# Autodesk Inventor assembly: Jar Jar
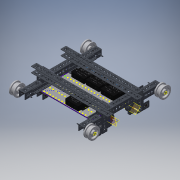
[picture p0: Inventor's stored thumbnail of the model, 180x180]
Saved by Autodesk Inventor 2016 (Build 200138000, 138)
## iProperties
Created: 2015-12-13
Part Number: Jar Jar
Document SubType Name: Assembly
Designer: tbloo
Author: tbloo
## Documents named in this file (17)
- C:\Users\TimB\Documents\GitHub\phi_robotics\3d-models\FTC_Tetrix_KOP_Block_Party\Tim Bloot Designs\JAr JaR Bot\Jar Jar.iam
- C:\Users\TimB\Documents\GitHub\phi_robotics\3d-models\FTC_Tetrix_KOP_Block_Party\Tim Bloot Designs\Base Plate.ipt
- C:\Users\TimB\Documents\GitHub\phi_robotics\3d-models\FTC_Tetrix_KOP_Block_Party\Tetrix_Kit_FTC\Autodesk Inventor Files\tetrix_c_channel-3.ipt
- C:\Users\TimB\Documents\GitHub\phi_robotics\3d-models\FTC_Tetrix_KOP_Block_Party\Tetrix_Kit_FTC\Autodesk Inventor Files\tetrix_c_channel-2.ipt
- C:\Users\TimB\Documents\GitHub\phi_robotics\3d-models\FTC_Tetrix_KOP_Block_Party\Tetrix_Kit_FTC\Autodesk Inventor Files\tetrix_motor_mount-old.ipt
- C:\Users\TimB\Documents\GitHub\phi_robotics\3d-models\FTC_Tetrix_KOP_Block_Party\Tetrix_Kit_FTC\Autodesk Inventor Files\tetrix_739274_2013.ipt
- C:\Users\TimB\Documents\GitHub\phi_robotics\3d-models\FTC_Tetrix_KOP_Block_Party\Tetrix_Kit_FTC\Autodesk Inventor Files\tetrix_motor.iam
- C:\Users\TimB\Documents\GitHub\phi_robotics\3d-models\FTC_Tetrix_KOP_Block_Party\Tetrix_Kit_FTC\Autodesk Inventor Files\tetrix_bushing.ipt
- C:\Users\TimB\Documents\GitHub\phi_robotics\3d-models\FTC_Tetrix_KOP_Block_Party\Tim Bloot Designs\JAr JaR Bot\Tread Wheel Assembly.iam
- C:\Users\TimB\Documents\GitHub\phi_robotics\3d-models\FTC_Tetrix_KOP_Block_Party\Tim Bloot Designs\JAr JaR Bot\tetrix_angle-144 MM.ipt
- C:\Users\TimB\Documents\GitHub\phi_robotics\3d-models\FTC_Tetrix_KOP_Block_Party\Tetrix_Kit_FTC\Autodesk Inventor Files\tetrix_c_channel-5.ipt
- C:\Users\TimB\Documents\GitHub\phi_robotics\3d-models\FTC_Tetrix_KOP_Block_Party\Tetrix_Kit_FTC\Autodesk Inventor Files\tetrix_inside_corner_bracket.ipt
- C:\Users\TimB\Documents\GitHub\phi_robotics\3d-models\FTC_Tetrix_KOP_Block_Party\Tetrix_Kit_FTC\Autodesk Inventor Files\tetrix_motor_controller.ipt
- C:\Users\TimB\Documents\GitHub\phi_robotics\3d-models\FTC_Tetrix_KOP_Block_Party\Tetrix_Kit_FTC\Autodesk Inventor Files\tetrix_servo_controller.ipt
- C:\Users\TimB\Documents\GitHub\phi_robotics\3d-models\FTC_Tetrix_KOP_Block_Party\Tetrix_Kit_FTC\Autodesk Inventor Files\tetrix_c_channel-round.ipt
- C:\Users\TimB\Documents\GitHub\phi_robotics\3d-models\FTC_Tetrix_KOP_Block_Party\Tetrix_Kit_FTC\Autodesk Inventor Files\tetrix_c_channel-1.ipt
- C:\Users\TimB\Documents\GitHub\phi_robotics\3d-models\FTC_Tetrix_KOP_Block_Party\Tetrix_Kit_FTC\Autodesk Inventor Files\tetrix_angle-288 MM.ipt
## Components (48 placed, 16 different names)
1. Base Plate:1 — Rigid:40, Rigid:60, Rigid:61, Rigid:63
2. tetrix_c_channel-3:3 — Rigid:37, Rigid:39, Rigid:54, Rigid:57
3. tetrix_c_channel-2:9
4. tetrix_c_channel-2:10
5. tetrix_c_channel-2:11 — Rigid:38
6. tetrix_c_channel-2:12 — Rigid:36
7. tetrix_motor_mount-old:3
8. tetrix_motor_mount-old:4
9. tetrix_739274_2013:3
10. tetrix_739274_2013:4
11. tetrix_motor:3 [sub-assembly]
12. tetrix_motor:4 [sub-assembly]
13. tetrix_bushing:5
14. tetrix_bushing:6
15. tetrix_bushing:7
16. tetrix_bushing:8
17. Tread Wheel Assembly:3 [sub-assembly]
18. Tread Wheel Assembly:4 [sub-assembly]
19. tetrix_angle-144 MM:1 — Rigid:36, Rigid:37, Rigid:40
20. tetrix_angle-144 MM:2 — Rigid:38, Rigid:39
21. tetrix_c_channel-3:4 — Rigid:55, Rigid:56, Rigid:76
22. tetrix_c_channel-2:13 — Rigid:64, Rotational:40
23. tetrix_c_channel-2:15
24. tetrix_c_channel-2:16
25. tetrix_motor_mount-old:6
26. tetrix_motor:5 [sub-assembly]
27. Tread Wheel Assembly:5 [sub-assembly]
28. Tread Wheel Assembly:6 [sub-assembly]
29. tetrix_c_channel-5:1 — Rigid:54, Rigid:55
30. tetrix_c_channel-5:2 — Rigid:58, Rigid:59
31. tetrix_inside_corner_bracket:1 — Rigid:57, Rigid:58
32. tetrix_inside_corner_bracket:2 — Rigid:56, Rigid:59
33. tetrix_motor_controller:1 — Rigid:61, Rigid:62
34. tetrix_motor_controller:2 — Rigid:60
35. tetrix_motor_controller:3 — Rigid:62
36. tetrix_servo_controller:1 — Rigid:63
37. tetrix_c_channel-round:1 — Rigid:64, Rigid:65
38. tetrix_c_channel-1:1 — Rigid:65, Rotational:33, Rotational:34
39. tetrix_bushing:13 — Rotational:33
40. tetrix_bushing:14 — Rotational:34
41. tetrix_c_channel-2:18 — Rigid:75
42. tetrix_motor_mount-old:8 — Rotational:41
43. tetrix_c_channel-round:3
44. tetrix_c_channel-1:3
45. tetrix_bushing:17
46. tetrix_bushing:18
47. tetrix_angle-288 MM:2 — Rotational:40, Rigid:75, Rigid:76
48. tetrix_motor:6 [sub-assembly] — Rotational:41
## Relationships (46: WeldJoint 29, RevoluteJoint 17)
- [WeldJoint]: tetrix_c_channel-2:9 ↔ tetrix_motor_mount-old:4
- [WeldJoint]: tetrix_c_channel-2:10 ↔ tetrix_motor_mount-old:3
- [WeldJoint]: tetrix_c_channel-2:9 ↔ tetrix_739274_2013:3
- [WeldJoint]: tetrix_c_channel-2:11 ↔ tetrix_739274_2013:3
- [WeldJoint]: tetrix_c_channel-2:10 ↔ tetrix_739274_2013:4
- [WeldJoint]: tetrix_c_channel-2:12 ↔ tetrix_739274_2013:4
- [RevoluteJoint]: tetrix_motor_mount-old:4 ↔ tetrix_motor:3
- [RevoluteJoint]: tetrix_motor_mount-old:3 ↔ tetrix_motor:4
- [RevoluteJoint]: tetrix_c_channel-2:9 ↔ tetrix_bushing:6
- [RevoluteJoint]: tetrix_c_channel-2:9 ↔ tetrix_bushing:5
- [RevoluteJoint]: tetrix_c_channel-2:10 ↔ tetrix_bushing:7
- [RevoluteJoint]: tetrix_c_channel-2:10 ↔ tetrix_bushing:8
- [RevoluteJoint]: tetrix_c_channel-2:11 ↔ Tread Wheel Assembly:3
- [RevoluteJoint]: tetrix_c_channel-2:12 ↔ Tread Wheel Assembly:4
- Rigid:36 [WeldJoint]: tetrix_c_channel-2:12 ↔ tetrix_angle-144 MM:1
- Rigid:37 [WeldJoint]: tetrix_c_channel-3:3 ↔ tetrix_angle-144 MM:1
- Rigid:38 [WeldJoint]: tetrix_c_channel-2:11 ↔ tetrix_angle-144 MM:2
- Rigid:39 [WeldJoint]: tetrix_c_channel-3:3 ↔ tetrix_angle-144 MM:2
- Rigid:40 [WeldJoint]: Base Plate:1 ↔ tetrix_angle-144 MM:1
- [WeldJoint]: tetrix_c_channel-2:13 ↔ tetrix_motor_mount-old:6
- [RevoluteJoint]: tetrix_motor_mount-old:6 ↔ tetrix_motor:5
- [RevoluteJoint]: tetrix_c_channel-2:15 ↔ Tread Wheel Assembly:5
- [RevoluteJoint]: tetrix_c_channel-2:16 ↔ Tread Wheel Assembly:6
- Rigid:54 [WeldJoint]: tetrix_c_channel-3:3 ↔ tetrix_c_channel-5:1
- Rigid:55 [WeldJoint]: tetrix_c_channel-3:4 ↔ tetrix_c_channel-5:1
- Rigid:56 [WeldJoint]: tetrix_c_channel-3:4 ↔ tetrix_inside_corner_bracket:2
- Rigid:57 [WeldJoint]: tetrix_c_channel-3:3 ↔ tetrix_inside_corner_bracket:1
- Rigid:58 [WeldJoint]: tetrix_c_channel-5:2 ↔ tetrix_inside_corner_bracket:1
- Rigid:59 [WeldJoint]: tetrix_c_channel-5:2 ↔ tetrix_inside_corner_bracket:2
- Rigid:60 [WeldJoint]: Base Plate:1 ↔ tetrix_motor_controller:2
- Rigid:61 [WeldJoint]: Base Plate:1 ↔ tetrix_motor_controller:1
- Rigid:62 [WeldJoint]: tetrix_motor_controller:1 ↔ tetrix_motor_controller:3
- Rigid:63 [WeldJoint]: Base Plate:1 ↔ tetrix_servo_controller:1
- Rigid:64 [WeldJoint]: tetrix_c_channel-2:13 ↔ tetrix_c_channel-round:1
- Rigid:65 [WeldJoint]: tetrix_c_channel-round:1 ↔ tetrix_c_channel-1:1
- Rotational:33 [RevoluteJoint]: tetrix_c_channel-1:1 ↔ tetrix_bushing:13
- Rotational:34 [RevoluteJoint]: tetrix_c_channel-1:1 ↔ tetrix_bushing:14
- [WeldJoint]: tetrix_c_channel-2:18 ↔ tetrix_motor_mount-old:8
- [WeldJoint]: tetrix_c_channel-2:18 ↔ tetrix_c_channel-round:3
- [WeldJoint]: tetrix_c_channel-round:3 ↔ tetrix_c_channel-1:3
- [RevoluteJoint]: tetrix_c_channel-1:3 ↔ tetrix_bushing:17
- [RevoluteJoint]: tetrix_c_channel-1:3 ↔ tetrix_bushing:18
- Rotational:40 [RevoluteJoint]: tetrix_c_channel-2:13 ↔ tetrix_angle-288 MM:2
- Rigid:75 [WeldJoint]: tetrix_c_channel-2:18 ↔ tetrix_angle-288 MM:2
- Rigid:76 [WeldJoint]: tetrix_c_channel-3:4 ↔ tetrix_angle-288 MM:2
- Rotational:41 [RevoluteJoint]: tetrix_motor_mount-old:8 ↔ tetrix_motor:6
## Named parameters: d46_d27 = 0 mm, d47_d28 = 4.697383 deg, d48_d29 = 0 mm, d49_d30 = 0.338188 deg, d52_d33 = 0 mm, d53_d34 = 0.814021 deg, d54_d35 = 0 mm, d55_d36 = -29.078357 deg, d58_d39 = 0 mm, d59_d40 = -5.431137 deg, d60_d41 = 0 mm, d61_d42 = 0.840635 deg, d65_d11 = 0 mm, d66_d12 = 0 mm, d67_d13 = 0 mm, d68_d14 = 0 mm, d69_d15 = 0 mm, d70_d16 = 0 mm, d71_d21 = 0 mm, d72_d22 = -9.167541 deg, d73_d23 = 0 mm, d74_d24 = -19.058032 deg, d112_d58_d39 = 0 mm, d113_d59_d40 = -5.431137 deg, d114_d60_d41 = 0 mm, d115_d61_d42 = 0.840635 deg, d116_d65_d11 = 0 mm, d122_d71_d21 = 0 mm, d123_d72_d22 = -45.624239 deg, d153_d150_d116_d65_d11 = 0 mm, d154_d143_d137 = 0 mm, d155_d144_d138 = 0 mm, d156_d145_d139 = 0 mm, d157_d146_d140 = 0 deg, d158_d147_d141 = 0 mm, d159_d148_d142 = 0 deg
